# Autodesk Inventor assembly: Frame 1647030135921
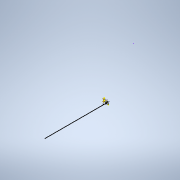
[picture p0: Inventor's stored thumbnail of the model, 180x180]
Saved by Autodesk Inventor 2022.2 (Build 262287010, 287A)
## iProperties
_FrameDoc: Frame Assembly
_Version: 25.0.0
Created: 2022-03-11
Part Number: Frame 1647030135921
Document SubType Name: Assembly
Designer: foriw
Mass: 3267.05 g
Surface Area: 4067.66 cm^2
Volume: 419.019 cm^3
Density: 7.79691 g/cm^3
Author: foriw
## Documents named in this file (28)
- C:\Users\Finn Oriwohl\Documents\htx\1g g\BeerCart-CAD-Inventor\Workspaces\Workspace\beercart assembly - mekatronik\Frame\Frame 1647030135921.iam
- C:\Users\Finn Oriwohl\Documents\htx\1g g\BeerCart-CAD-Inventor\Workspaces\Workspace\beercart assembly - mekatronik\Frame\Skeleton 1647030135922.ipt
- C:\Users\Finn Oriwohl\Documents\htx\1g g\BeerCart-CAD-Inventor\Workspaces\Workspace\beercart assembly - mekatronik\Frame\ISO 12633-2 20x20x2 1647030137505.ipt
- C:\Users\Finn Oriwohl\Documents\htx\1g g\BeerCart-CAD-Inventor\Workspaces\Workspace\beercart assembly - mekatronik\Frame\ISO 12633-2 20x20x2 1647030138110.ipt
- C:\Users\Finn Oriwohl\Documents\htx\1g g\BeerCart-CAD-Inventor\Workspaces\Workspace\beercart assembly - mekatronik\Frame\ISO 12633-2 20x20x2 1647030138225.ipt
- C:\Users\Finn Oriwohl\Documents\htx\1g g\BeerCart-CAD-Inventor\Workspaces\Workspace\beercart assembly - mekatronik\Frame\ISO 12633-2 20x20x2 1647030639616.ipt
- C:\Users\Finn Oriwohl\Documents\htx\1g g\BeerCart-CAD-Inventor\Workspaces\Workspace\beercart assembly - mekatronik\Frame\ISO 12633-2 20x20x2 1647030639707.ipt
- C:\Users\Finn Oriwohl\Documents\htx\1g g\BeerCart-CAD-Inventor\Workspaces\Workspace\beercart assembly - mekatronik\Frame\ISO 1035_2 10x 10 1647602096505.ipt
- C:\Users\Finn Oriwohl\Documents\htx\1g g\BeerCart-CAD-Inventor\Workspaces\Workspace\beercart assembly - mekatronik\Frame\ISO 1035_2 10x 10 1647602096566.ipt
- C:\Users\Finn Oriwohl\Documents\htx\1g g\BeerCart-CAD-Inventor\Workspaces\Workspace\beercart assembly - mekatronik\Frame\ISO 1035_2 10x 10 1647602096620.ipt
- C:\Users\Finn Oriwohl\Documents\htx\1g g\BeerCart-CAD-Inventor\Workspaces\Workspace\beercart assembly - mekatronik\Frame\ISO 12633-2 20x20x2 1647606177319.ipt
- C:\Users\Finn Oriwohl\Documents\htx\1g g\BeerCart-CAD-Inventor\Workspaces\Workspace\beercart assembly - mekatronik\Frame\ISO 12633-2 20x20x2 1647606177438.ipt
- C:\Users\Finn Oriwohl\Documents\htx\1g g\BeerCart-CAD-Inventor\Workspaces\Workspace\beercart assembly - mekatronik\Frame\FrontWheelFrame.iam
- C:\Users\Finn Oriwohl\Documents\htx\1g g\BeerCart-CAD-Inventor\Workspaces\Workspace\BackWheelMountingPlate.ipt
- C:\Users\Finn Oriwohl\Documents\htx\1g g\BeerCart-CAD-Inventor\Workspaces\Workspace\BackWheelMountingPlate_MIR_MIR.ipt
- C:\Users\Finn Oriwohl\Documents\htx\1g g\BeerCart-CAD-Inventor\Workspaces\Workspace\beercart assembly - mekatronik\Frame\ISO 1035_2 10x 10 1648211737860.ipt
- C:\Users\Finn Oriwohl\Documents\htx\1g g\BeerCart-CAD-Inventor\Workspaces\Workspace\bearing housing front.ipt
- C:\Users\Finn Oriwohl\Documents\htx\1g g\BeerCart-CAD-Inventor\Workspaces\Workspace\beercart assembly - mekatronik\Frame\ISO 12633-2 20x20x2 1648573909221.ipt
- C:\Users\Finn Oriwohl\Documents\htx\1g g\BeerCart-CAD-Inventor\Workspaces\Workspace\beercart assembly - mekatronik\Frame\ISO 12633-2 20x20x2 1648573975084.ipt
- C:\Users\Finn Oriwohl\Documents\htx\1g g\BeerCart-CAD-Inventor\Workspaces\Workspace\beercart assembly - mekatronik\Frame\ISO 12633-2 20x20x2 1648627088055.ipt
- C:\Users\Finn Oriwohl\Documents\htx\1g g\BeerCart-CAD-Inventor\Workspaces\Workspace\beercart assembly - mekatronik\Frame\ISO 12633-2 20x20x2 1648627088175.ipt
- C:\Users\Finn Oriwohl\Documents\htx\1g g\BeerCart-CAD-Inventor\Workspaces\Workspace\BackWheelMountingPlate_MIR4.ipt
- C:\Users\Finn Oriwohl\Documents\htx\1g g\BeerCart-CAD-Inventor\Workspaces\Workspace\beercart assembly - mekatronik\Frame\ISO 12633-2 20x20x2 1648631331581.ipt
- C:\Users\Finn Oriwohl\Documents\htx\1g g\BeerCart-CAD-Inventor\Workspaces\Workspace\beercart assembly - mekatronik\Frame\ISO 12633-2 20x20x2 1649085652950.ipt
- C:\Users\Finn Oriwohl\Documents\htx\1g g\BeerCart-CAD-Inventor\Workspaces\Workspace\beercart assembly - mekatronik\Frame\ISO 12633-2 20x20x2 1649085653040.ipt
- C:\Users\Finn Oriwohl\Documents\htx\1g g\BeerCart-CAD-Inventor\Workspaces\Workspace\backWheelNoMotor brake mount.ipt
- C:\Users\Finn Oriwohl\Documents\htx\1g g\BeerCart-CAD-Inventor\Workspaces\Workspace\beercart assembly - mekatronik\Frame\ISO 12633-2 20x20x2 1649154464355.ipt
- C:\Users\Finn Oriwohl\Documents\htx\1g g\BeerCart-CAD-Inventor\Workspaces\Workspace\BackWheelMotorMountSpacer.ipt
## Components (27 placed, 22 different names)
1. bearing housing front:1 — Rotational:1
2. Reference Skeleton
3. ISO 12633-2 20x20x2 - 319,95:2
4. ISO 12633-2 20x20x2 - 290:1
5. ISO 12633-2 20x20x2 - 159.94:3
6. ISO 12633-2 20x20x2 - 182.18:1
7. ISO 12633-2 20x20x2 - 182.18:2
8. ISO 1035/2 10x 10 - 58.08:1
9. ISO 1035/2 10x 10 - 68.33:1
10. ISO 1035/2 10x 10 - 68.33:2
11. ISO 12633-2 20x20x2 - 152.97:1 — Mate:1, Mate:3
12. ISO 12633-2 20x20x2 - 152.97:2 — Mate:2, Mate:4, Mate:5
13. BackWheelMountingPlate:1 — Flush:6, Rotational:2, Rigid:1
14. FrontWheelFrame:1 [sub-assembly] — Rotational:1
15. BackWheelMountingPlate_MIR_MIR:1
16. ISO 1035/2 10x 10 - 58.08:1
17. ISO 12633-2 20x20x2 - 277.56:1
18. ISO 12633-2 20x20x2 - 44,58:1 — Flush:6, Rotational:2, Rigid:1
19. ISO 12633-2 20x20x2 - 33,46:1 — Rotational:5, Flush:9, Flush:11, Flush:12, Flush:13
20. ISO 12633-2 20x20x2 - 98,7:1
21. BackWheelMountingPlate_MIR4:1 — Rotational:5, Flush:9
22. ISO 12633-2 20x20x2 - 290,25:1
23. ISO 12633-2 20x20x2 - 98.7:1
24. ISO 12633-2 20x20x2 - 33,46:1 — Flush:10
25. backWheelNoMotor brake mount:1 — Flush:10
26. ISO 12633-2 20x20x2 - 44.58:1
27. BackWheelMotorMountSpacer:1 — Flush:11, Flush:12, Flush:13
## Relationships (17: Flush 7, Mate 6, RevoluteJoint 3, WeldJoint 1)
- Mate:1: ISO 12633-2 20x20x2 - 152.97:1
- Mate:2: ISO 12633-2 20x20x2 - 152.97:2
- Mate:3: ISO 12633-2 20x20x2 - 152.97:1
- Mate:4: ISO 12633-2 20x20x2 - 152.97:2
- Mate:5: ISO 12633-2 20x20x2 - 152.97:2
- [Mate]: bearing housing front:1 ↔ ISO 1035/2 10x 10 - 58.08:1
- [Flush] (1 mm): bearing housing front:1 ↔ ISO 1035/2 10x 10 - 58.08:1
- Rotational:1 [RevoluteJoint] (4 mm): bearing housing front:1 ↔ FrontWheelFrame:1
- Flush:6: BackWheelMountingPlate:1 ↔ ISO 12633-2 20x20x2 - 44,58:1
- Rotational:2 [RevoluteJoint]: BackWheelMountingPlate:1 ↔ ISO 12633-2 20x20x2 - 44,58:1
- Rotational:5 [RevoluteJoint]: ISO 12633-2 20x20x2 - 33,46:1 ↔ BackWheelMountingPlate_MIR4:1
- Flush:9: ISO 12633-2 20x20x2 - 33,46:1 ↔ BackWheelMountingPlate_MIR4:1
- Flush:10: ISO 12633-2 20x20x2 - 33,46:1 ↔ backWheelNoMotor brake mount:1
- Rigid:1 [WeldJoint]: BackWheelMountingPlate:1 ↔ ISO 12633-2 20x20x2 - 44,58:1
- Flush:11: ISO 12633-2 20x20x2 - 33,46:1 ↔ BackWheelMotorMountSpacer:1
- Flush:12: ISO 12633-2 20x20x2 - 33,46:1 ↔ BackWheelMotorMountSpacer:1
- Flush:13: ISO 12633-2 20x20x2 - 33,46:1 ↔ BackWheelMotorMountSpacer:1
## Named parameters: d22_d2 = 0 mm, d23_d3 = 1 mm
